# Autodesk Inventor assembly: Ensamblaje
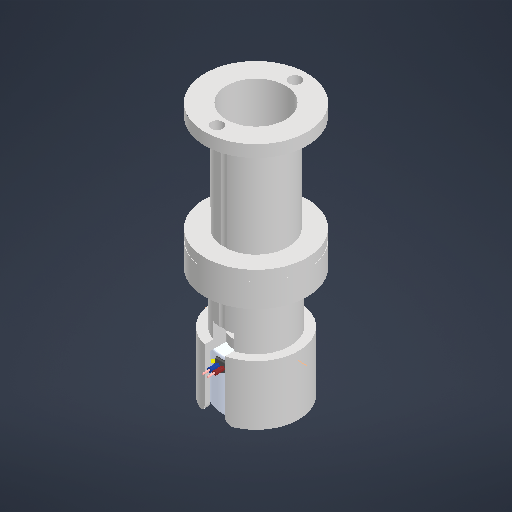
[picture p0: Inventor's stored thumbnail of the model, 512x512]
Saved by Autodesk Inventor 2026.3 (Build 303398000, 398)
## iProperties
Created: 2026-07-22
Part Number: Ensamblaje
Document SubType Name: Assembly
Designer: ASUS
Author: ASUS
## Documents named in this file (5)
- C:\Users\ASUS\Desktop\Robótica\Proyecto\Soporte\Ensamblaje.iam
- C:\Users\ASUS\Desktop\Robótica\Proyecto\Soporte\-electromagnet-customsize-collection\20-15 (2.5kg 12V).ipt
- C:\Users\ASUS\Desktop\Robótica\Proyecto\Robot\epson_t3_401s_step\Primer parte.ipt
- C:\Users\ASUS\Desktop\Robótica\Proyecto\Robot\epson_t3_401s_step\SegundaParte.ipt
- C:\Users\ASUS\Desktop\Robótica\Proyecto\Robot\epson_t3_401s_step\TeceraParte.ipt
## Components (4 placed, 4 different names)
1. 20-15 (2.5kg 12V):1 — Nivelación:4
2. Primer parte:1 — Nivelación:3, Nivelación:4
3. SegundaParte:1 — Nivelación:3, Coincidencia:3
4. TeceraParte:1 — Coincidencia:3
## Relationships (3: Flush 2, Mate 1)
- Nivelación:3 [Flush]: Primer parte:1 ↔ SegundaParte:1
- Nivelación:4 [Flush]: 20-15 (2.5kg 12V):1 ↔ Primer parte:1
- Coincidencia:3 [Mate]: SegundaParte:1 ↔ TeceraParte:1
